# Autodesk Inventor assembly: bras
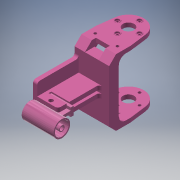
[picture p0: Inventor's stored thumbnail of the model, 180x180]
Saved by Autodesk Inventor 2019 (Build 230136000, 136)
## iProperties
Created: 2020-02-16
Part Number: bras
Document SubType Name: Assembly
Designer: franc
Author: franc
## Documents named in this file (3)
- C:\Users\franc\Desktop\EsialRobotik\Mecanique\2020\pmi\bras.iam
- C:\Users\franc\Desktop\EsialRobotik\Mecanique\2020\pmi\supportTestVentouse.ipt
- C:\Users\franc\Desktop\EsialRobotik\Mecanique\2020\pmi\F2.ipt
## Components (2 placed, 2 different names)
1. supportTestVentouse:1 — Placage:1, Placage:2
2. F2:1 — Placage:1, Placage:2
## Relationships (2: Mate 2)
- Placage:1 [Mate]: supportTestVentouse:1 ↔ F2:1
- Placage:2 [Mate]: supportTestVentouse:1 ↔ F2:1
